# Autodesk Inventor assembly: camaAssem1-RP1
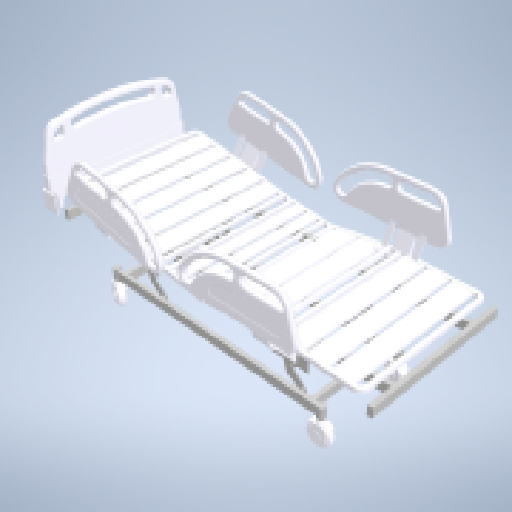
[picture p0: Inventor's stored thumbnail of the model, 512x512]
Saved by Autodesk Inventor 2023 (Build 270158000, 158)
## iProperties
Created: 2022-03-28
Part Number: camaAssem1-RP1
Document SubType Name: Assembly
Designer: klebe
Sending System: SolidWorks 2017
Last Author: MUSTOFA
Last Saved: 2022-03-28
Author: klebe
## Documents named in this file (15)
- C:\Users\klebe\OneDrive\Documents\GitHub\Sala-braquiterapia\Sala de Braquiterapia\Inventor\hospital-bed-ranjang-pasien-tempat-tidur-pasien-1.snapshot.4\cama\camaAssem1-RP1.iam
- C:\Users\klebe\OneDrive\Documents\GitHub\Sala-braquiterapia\Sala de Braquiterapia\Inventor\hospital-bed-ranjang-pasien-tempat-tidur-pasien-1.snapshot.4\camaRP1-1.ipt
- C:\Users\klebe\OneDrive\Documents\GitHub\Sala-braquiterapia\Sala de Braquiterapia\Inventor\hospital-bed-ranjang-pasien-tempat-tidur-pasien-1.snapshot.4\camaRP1-7.ipt
- C:\Users\klebe\OneDrive\Documents\GitHub\Sala-braquiterapia\Sala de Braquiterapia\Inventor\hospital-bed-ranjang-pasien-tempat-tidur-pasien-1.snapshot.4\camaRP1-8.ipt
- C:\Users\klebe\OneDrive\Documents\GitHub\Sala-braquiterapia\Sala de Braquiterapia\Inventor\hospital-bed-ranjang-pasien-tempat-tidur-pasien-1.snapshot.4\camaRP1-2.ipt
- C:\Users\klebe\OneDrive\Documents\GitHub\Sala-braquiterapia\Sala de Braquiterapia\Inventor\hospital-bed-ranjang-pasien-tempat-tidur-pasien-1.snapshot.4\camaRP1-3.ipt
- C:\Users\klebe\OneDrive\Documents\GitHub\Sala-braquiterapia\Sala de Braquiterapia\Inventor\hospital-bed-ranjang-pasien-tempat-tidur-pasien-1.snapshot.4\camaRP1-4.ipt
- C:\Users\klebe\OneDrive\Documents\GitHub\Sala-braquiterapia\Sala de Braquiterapia\Inventor\hospital-bed-ranjang-pasien-tempat-tidur-pasien-1.snapshot.4\camaRP1-5.ipt
- C:\Users\klebe\OneDrive\Documents\GitHub\Sala-braquiterapia\Sala de Braquiterapia\Inventor\hospital-bed-ranjang-pasien-tempat-tidur-pasien-1.snapshot.4\camaRP1-6.ipt
- C:\Users\klebe\OneDrive\Documents\GitHub\Sala-braquiterapia\Sala de Braquiterapia\Inventor\hospital-bed-ranjang-pasien-tempat-tidur-pasien-1.snapshot.4\camahead board-RP1.ipt
- C:\Users\klebe\OneDrive\Documents\GitHub\Sala-braquiterapia\Sala de Braquiterapia\Inventor\hospital-bed-ranjang-pasien-tempat-tidur-pasien-1.snapshot.4\camaRP1-BT-1-A.ipt
- C:\Users\klebe\OneDrive\Documents\GitHub\Sala-braquiterapia\Sala de Braquiterapia\Inventor\hospital-bed-ranjang-pasien-tempat-tidur-pasien-1.snapshot.4\camaRP1-BT-1-B.ipt
- C:\Users\klebe\OneDrive\Documents\GitHub\Sala-braquiterapia\Sala de Braquiterapia\Inventor\hospital-bed-ranjang-pasien-tempat-tidur-pasien-1.snapshot.4\cama\Part25.ipt
- C:\Users\klebe\OneDrive\Documents\GitHub\Sala-braquiterapia\Sala de Braquiterapia\Inventor\hospital-bed-ranjang-pasien-tempat-tidur-pasien-1.snapshot.4\cama\Part61.ipt
- C:\Users\klebe\OneDrive\Documents\GitHub\Sala-braquiterapia\Sala de Braquiterapia\Inventor\hospital-bed-ranjang-pasien-tempat-tidur-pasien-1.snapshot.4\Part62.ipt
## Components (17 placed, 14 different names)
1. RP1-1:1 — Flush:6, Flush:7
2. RP1-7:1
3. RP1-7:2
4. RP1-8:1
5. RP1-8:2
6. RP1-2:1 — Flush:1, Mate:1, Flush:5, Rigid:3
7. RP1-3:1 — Rotational:3, Rigid:1, Rigid:2
8. RP1-4:1 — Rotational:2, Rotational:3, Flush:1, Mate:1, Mate:2
9. RP1-5:1 — Rotational:2, Rotational:4, Mate:2, Mate:3, Flush:2, Flush:3
10. RP1-6:1 — Rotational:4, Mate:3
11. head board-RP1:2
12. RP1-BT-1-A:2 — Rigid:2
13. RP1-BT-1-B:2 — Rigid:1
14. Part25:1 — Flush:2, Flush:3, Flush:4
15. Part61:1 — Flush:4, Flush:5
16. Part61:2 — Rigid:3
17. Part62:1 — Flush:6, Flush:7
## Relationships (16: Flush 7, RevoluteJoint 3, WeldJoint 3, Mate 3)
- Rotational:2 [RevoluteJoint]: RP1-4:1 ↔ RP1-5:1
- Rotational:3 [RevoluteJoint]: RP1-3:1 ↔ RP1-4:1
- Rotational:4 [RevoluteJoint]: RP1-5:1 ↔ RP1-6:1
- Rigid:1 [WeldJoint]: RP1-3:1 ↔ RP1-BT-1-B:2
- Rigid:2 [WeldJoint]: RP1-3:1 ↔ RP1-BT-1-A:2
- Flush:1: RP1-2:1 ↔ RP1-4:1
- Mate:1: RP1-2:1 ↔ RP1-4:1
- Mate:2: RP1-4:1 ↔ RP1-5:1
- Mate:3: RP1-5:1 ↔ RP1-6:1
- Flush:2: RP1-5:1 ↔ Part25:1
- Flush:3: RP1-5:1 ↔ Part25:1
- Flush:4: Part25:1 ↔ Part61:1
- Flush:5: RP1-2:1 ↔ Part61:1
- Rigid:3 [WeldJoint]: RP1-2:1 ↔ Part61:2
- Flush:6: RP1-1:1 ↔ Part62:1
- Flush:7: RP1-1:1 ↔ Part62:1
